# Autodesk Inventor assembly: GAME ELEMENT FINAL
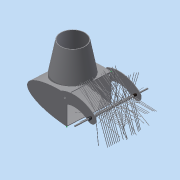
[picture p0: Inventor's stored thumbnail of the model, 180x180]
Saved by Autodesk Inventor 2015 (Build 190159000, 159)
## iProperties
Created: 2014-09-21
Part Number: GAME ELEMENT FINAL
Document SubType Name: Assembly
Designer: Kris
Author: Kris
## Documents named in this file (7)
- C:\Working Folder\CAD Models\GAME ELEMENT FINAL.iam
- C:\Working Folder\CAD Models\Long Axle 250mm.ipt
- C:\Working Folder\CAD Models\tetrix_739091_2013.ipt
- C:\Working Folder\CAD Models\tetrix_739092_2012.iam
- C:\Working Folder\CAD Models\Fan System.iam
- C:\Working Folder\CAD Models\Game.ipt
- C:\Working Folder\CAD Models\Cannon.ipt
## Components (30 placed, 6 different names)
1. tetrix_739091_2013:1 — Mate:11, Mate:75, Mate:76, Mate:79
2. tetrix_739091_2013:2 — Mate:16, Mate:66, Mate:67, Mate:77, Mate:78
3. tetrix_739092_2012:1 [sub-assembly] — Mate:17, Mate:78
4. tetrix_739092_2012:2 [sub-assembly] — Mate:15, Mate:76
5. Long Axle 250mm:1 — Mate:11, Flush:3, Mate:13, Mate:15, Mate:16, Mate:17, Flush:5, Mate:18, Mate:21, Mate:23, Mate:25, Mate:27, Mate:29, Mate:31, Mate:33, Mate:35, Mate:37, Mate:39, Mate:41, Mate:43, Mate:44, Mate:47, Mate:49, Mate:51, Mate:53, Mate:55, Mate:57, Mate:59, Mate:63, Mate:66, Mate:67, Mate:70, Mate:85
6. Fan System:1 [sub-assembly] — Mate:33, Mate:34, Mate:36
7. Fan System:2 [sub-assembly] — Mate:41, Mate:42, Mate:45
8. Fan System:3 [sub-assembly] — Mate:29, Mate:30, Mate:32
9. Fan System:4 [sub-assembly] — Mate:18, Mate:20, Mate:22
10. Fan System:5 [sub-assembly] — Mate:13, Flush:6, Mate:20, Mate:85
11. Fan System:6 [sub-assembly] — Mate:43, Mate:46, Mate:48
12. Fan System:7 [sub-assembly] — Mate:31, Mate:32, Mate:34
13. Fan System:8 [sub-assembly] — Mate:35, Mate:36, Mate:38
14. Fan System:9 [sub-assembly] — Mate:23, Mate:24, Mate:26
15. Fan System:10 [sub-assembly] — Mate:44, Mate:45, Mate:46
16. Fan System:11 [sub-assembly] — Mate:25, Mate:26, Mate:28
17. Fan System:12 [sub-assembly] — Mate:21, Mate:22, Mate:24
18. Fan System:13 [sub-assembly] — Mate:27, Mate:28, Mate:30
19. Fan System:14 [sub-assembly] — Mate:37, Mate:38, Mate:40
20. Fan System:15 [sub-assembly] — Mate:39, Mate:40, Mate:42
21. Fan System:16 [sub-assembly] — Mate:51, Mate:52, Mate:54
22. Fan System:17 [sub-assembly] — Mate:49, Mate:50, Mate:52
23. Fan System:18 [sub-assembly] — Mate:53, Mate:54, Mate:56
24. Fan System:19 [sub-assembly] — Mate:47, Mate:48, Mate:50
25. Fan System:20 [sub-assembly] — Mate:55, Mate:56, Mate:58
26. Fan System:21 [sub-assembly] — Mate:57, Mate:58, Mate:60
27. Fan System:22 [sub-assembly] — Mate:59, Mate:60, Mate:79
28. Game:1 — Flush:8, Mate:72, Mate:74, Mate:81, Mate:82, Mate:83, Mate:84
29. Cannon:1 — Mate:63, Mate:74, Mate:75, Flush:9, Mate:83, Mate:84
30. Cannon:2 — Mate:70, Mate:72, Mate:77, Mate:81, Mate:82
## Relationships (71: Mate 66, Flush 5)
- Mate:2 (38.1 mm)
- Mate:11: tetrix_739091_2013:1 ↔ Long Axle 250mm:1
- Flush:3: Long Axle 250mm:1
- Mate:12 (38.1 mm)
- Mate:13: Long Axle 250mm:1 ↔ Fan System:5
- Mate:15: tetrix_739092_2012:2 ↔ Long Axle 250mm:1
- Mate:16: tetrix_739091_2013:2 ↔ Long Axle 250mm:1
- Mate:17: tetrix_739092_2012:1 ↔ Long Axle 250mm:1
- Flush:5: Long Axle 250mm:1
- Mate:18: Long Axle 250mm:1 ↔ Fan System:4
- Flush:6 (22.86 mm): Fan System:5
- Mate:20 (4.572 mm): Fan System:4 ↔ Fan System:5
- Mate:21: Long Axle 250mm:1 ↔ Fan System:12
- Mate:22 (4.572 mm): Fan System:4 ↔ Fan System:12
- Mate:23: Long Axle 250mm:1 ↔ Fan System:9
- Mate:24 (4.572 mm): Fan System:9 ↔ Fan System:12
- Mate:25: Long Axle 250mm:1 ↔ Fan System:11
- Mate:26 (4.572 mm): Fan System:9 ↔ Fan System:11
- Mate:27: Long Axle 250mm:1 ↔ Fan System:13
- Mate:28 (4.572 mm): Fan System:11 ↔ Fan System:13
- Mate:29: Long Axle 250mm:1 ↔ Fan System:3
- Mate:30 (4.572 mm): Fan System:3 ↔ Fan System:13
- Mate:31: Long Axle 250mm:1 ↔ Fan System:7
- Mate:32 (4.572 mm): Fan System:3 ↔ Fan System:7
- Mate:33: Long Axle 250mm:1 ↔ Fan System:1
- Mate:34 (4.572 mm): Fan System:1 ↔ Fan System:7
- Mate:35: Long Axle 250mm:1 ↔ Fan System:8
- Mate:36 (4.572 mm): Fan System:1 ↔ Fan System:8
- Mate:37: Long Axle 250mm:1 ↔ Fan System:14
- Mate:38 (4.572 mm): Fan System:8 ↔ Fan System:14
- Mate:39: Long Axle 250mm:1 ↔ Fan System:15
- Mate:40 (4.572 mm): Fan System:14 ↔ Fan System:15
- Mate:41: Long Axle 250mm:1 ↔ Fan System:2
- Mate:42 (4.572 mm): Fan System:2 ↔ Fan System:15
- Mate:43: Long Axle 250mm:1 ↔ Fan System:6
- Mate:44: Long Axle 250mm:1 ↔ Fan System:10
- Mate:45 (4.572 mm): Fan System:2 ↔ Fan System:10
- Mate:46 (4.572 mm): Fan System:6 ↔ Fan System:10
- Mate:47: Long Axle 250mm:1 ↔ Fan System:19
- Mate:48 (4.572 mm): Fan System:6 ↔ Fan System:19
- Mate:49: Long Axle 250mm:1 ↔ Fan System:17
- Mate:50 (4.572 mm): Fan System:17 ↔ Fan System:19
- Mate:51: Long Axle 250mm:1 ↔ Fan System:16
- Mate:52 (4.572 mm): Fan System:16 ↔ Fan System:17
- Mate:53: Long Axle 250mm:1 ↔ Fan System:18
- Mate:54 (4.572 mm): Fan System:16 ↔ Fan System:18
- Mate:55: Long Axle 250mm:1 ↔ Fan System:20
- Mate:56 (4.572 mm): Fan System:18 ↔ Fan System:20
- Mate:57: Long Axle 250mm:1 ↔ Fan System:21
- Mate:58 (4.572 mm): Fan System:20 ↔ Fan System:21
- Mate:59: Long Axle 250mm:1 ↔ Fan System:22
- Mate:60 (4.572 mm): Fan System:21 ↔ Fan System:22
- Flush:8 (101.6 mm): Game:1
- Mate:63: Long Axle 250mm:1 ↔ Cannon:1
- Mate:66: tetrix_739091_2013:2 ↔ Long Axle 250mm:1
- Mate:67: tetrix_739091_2013:2 ↔ Long Axle 250mm:1
- Mate:70: Long Axle 250mm:1 ↔ Cannon:2
- Mate:72: Game:1 ↔ Cannon:2
- Mate:74: Game:1 ↔ Cannon:1
- Mate:75: tetrix_739091_2013:1 ↔ Cannon:1
- Mate:76: tetrix_739091_2013:1 ↔ tetrix_739092_2012:2
- Mate:77: tetrix_739091_2013:2 ↔ Cannon:2
- Mate:78: tetrix_739091_2013:2 ↔ tetrix_739092_2012:1
- Mate:79 (2.286 mm): tetrix_739091_2013:1 ↔ Fan System:22
- Flush:9: Cannon:1
- Mate:80 (38.1 mm)
- Mate:81: Game:1 ↔ Cannon:2
- Mate:82: Game:1 ↔ Cannon:2
- Mate:83: Game:1 ↔ Cannon:1
- Mate:84: Game:1 ↔ Cannon:1
- Mate:85: Long Axle 250mm:1 ↔ Fan System:5
